# Autodesk Inventor assembly: _arm
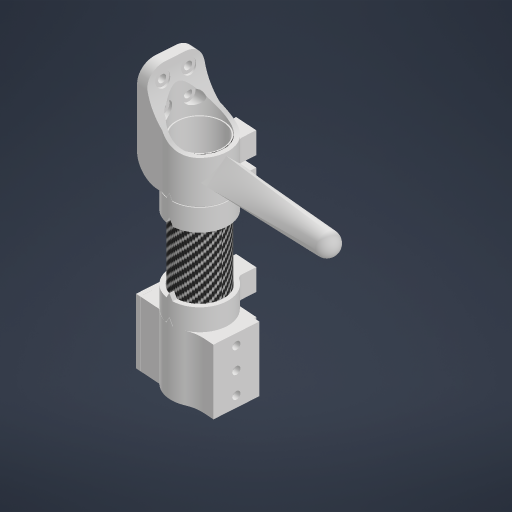
[picture p0: Inventor's stored thumbnail of the model, 512x512]
Saved by Autodesk Inventor 2023 (Build 270158000, 158)
## iProperties
Created: 2022-05-26
Part Number: _arm
Document SubType Name: Assembly
Designer: vibhu
Author: vibhu
## Documents named in this file (6)
- D:\Documents\_Personal\Projects\Drone\Drone\CAD\arm\_arm.iam
- D:\Documents\_Personal\Projects\Drone\Drone\CAD\arm\body holder.ipt
- D:\Documents\_Personal\Projects\Drone\Drone\CAD\arm\motor holder.ipt
- D:\Documents\_Personal\Projects\Drone\Drone\CAD\arm\tube.ipt
- D:\Documents\_Personal\Projects\Drone\Drone\CAD\arm\arm indexer 1cm.ipt
- D:\Documents\_Personal\Projects\Drone\Drone\CAD\arm\top spacer.ipt
## Components (6 placed, 5 different names)
1. body holder:1 — Mate:3, Flush:1, Angle:1, Mate:6, Flush:3, Flush:4, Flush:5
2. motor holder:1 — Mate:1, Mate:2, Angle:1, Mate:7, Flush:2
3. tube:1 — Mate:1, Mate:2, Mate:3, Flush:1, Mate:4, Mate:5
4. arm indexer 1cm:1 — Mate:5, Mate:6, Flush:3
5. arm indexer 1cm:2 — Mate:4, Mate:7, Flush:2
6. top spacer:1 — Flush:4, Flush:5
## Relationships (13: Mate 7, Flush 5, Angle 1)
- Mate:1: motor holder:1 ↔ tube:1
- Mate:2: motor holder:1 ↔ tube:1
- Mate:3: body holder:1 ↔ tube:1
- Flush:1: body holder:1 ↔ tube:1
- Angle:1 (0 deg): body holder:1 ↔ motor holder:1
- Mate:4: tube:1 ↔ arm indexer 1cm:2
- Mate:5: tube:1 ↔ arm indexer 1cm:1
- Mate:6: body holder:1 ↔ arm indexer 1cm:1
- Mate:7: motor holder:1 ↔ arm indexer 1cm:2
- Flush:2: motor holder:1 ↔ arm indexer 1cm:2
- Flush:3: body holder:1 ↔ arm indexer 1cm:1
- Flush:4: body holder:1 ↔ top spacer:1
- Flush:5: body holder:1 ↔ top spacer:1
